# Autodesk Inventor assembly: euph cart bottom
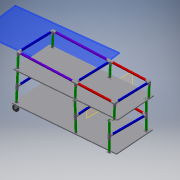
[picture p0: Inventor's stored thumbnail of the model, 180x180]
Saved by Autodesk Inventor 2018.2 (Build 222227000, 227)
## iProperties
Created: 2018-02-07
Part Number: euph cart bottom
Document SubType Name: Assembly
Designer: owner
Author: owner
## Documents named in this file (12)
- Z:\The Pickle\Final Carts\Euph Cart\euph cart bottom.iam
- Z:\The Pickle\Final Carts\Euph Cart\Plywood Base.ipt
- Z:\The Pickle\Inventor Pipe Parts\Formufit Fittings\4-way Tee 1 Inch.ipt
- Z:\The Pickle\Inventor Pipe Parts\Formufit Fittings\Tee 1 Inch.ipt
- Z:\The Pickle\Inventor Pipe Parts\Formufit Fittings\Wood Mount 1 Inch.ipt
- Z:\The Pickle\Final Carts\Euph Cart\Pipe 1.ipt
- Z:\The Pickle\Final Carts\Euph Cart\Pipe 2.ipt
- Z:\The Pickle\Final Carts\Euph Cart\Pipe 3.ipt
- Z:\The Pickle\Final Carts\WHEELS.ipt
- Z:\The Pickle\Final Carts\Mellie Cart\Pipe 4.ipt
- Z:\The Pickle\Inventor Pipe Parts\Formufit Fittings\5-way 1 Inch.ipt
- Z:\The Pickle\Inventor Pipe Parts\Formufit Fittings\3-way 90 1 Inch.ipt
## Components (65 placed, 11 different names)
1. Tee 1 Inch:4 — Insert:41, Insert:42, Insert:45
2. Pipe 1:2 — Insert:51, Insert:65
3. Plywood Base:2 — Mate:3, Flush:4, Flush:5, Flush:6, Tangent:6, Tangent:7, Flush:18, Flush:19, Mate:7
4. 4-way Tee 1 Inch:5
5. Wood Mount 1 Inch:9 — Tangent:6, Tangent:7, Flush:12, Mate:7
6. Wood Mount 1 Inch:10 — Flush:13
7. Wood Mount 1 Inch:11 — Flush:14
8. Wood Mount 1 Inch:12 — Flush:15
9. Pipe 1:3 — Insert:42
10. Pipe 2:4 — Insert:50
11. Pipe 3:9 — Insert:49
12. Pipe 3:10
13. Pipe 3:11 — Insert:41
14. Pipe 3:12 — Insert:72
15. Pipe 3:13 — Insert:52, Insert:73
16. Pipe 3:14 — Insert:66, Insert:74
17. Pipe 3:15 — Insert:45, Insert:71, Mate:6
18. Pipe 3:16 — Insert:70
19. WHEELS:1 — Flush:2, Flush:3, Mate:3, Flush:4, Flush:5, Flush:7
20. WHEELS:2 — Flush:2, Flush:6, Flush:7, Flush:11
21. WHEELS:4 — Flush:3, Flush:11
22. Pipe 4:3 — Insert:118, Insert:119
23. Pipe 4:7 — Insert:58
24. Pipe 1:11 — Insert:57, Insert:67
25. Wood Mount 1 Inch:13 — Insert:63, Flush:17
26. Wood Mount 1 Inch:14 — Insert:64, Flush:16
27. Wood Mount 1 Inch:15 — Insert:72, Flush:13
28. Wood Mount 1 Inch:16 — Insert:73, Flush:15
29. Wood Mount 1 Inch:17 — Insert:71, Flush:12, Mate:4
30. Wood Mount 1 Inch:18 — Insert:74, Flush:14
31. 5-way 1 Inch:1 — Insert:49, Insert:50, Insert:51, Insert:52
32. 4-way Tee 1 Inch:6 — Insert:57, Insert:58, Insert:61, Insert:62
33. Pipe 3:17 — Insert:63, Insert:68
34. Pipe 3:18 — Insert:69, Insert:75
35. Pipe 3:23 — Insert:61, Insert:64
36. Pipe 3:26 — Insert:62, Insert:76
37. Tee 1 Inch:5 — Insert:65, Insert:66, Insert:70
38. Tee 1 Inch:6 — Insert:67, Insert:68, Insert:69
39. Plywood Base:3 — Mate:4, Flush:18, Flush:19, Mate:5
40. Wood Mount 1 Inch:19 — Insert:75, Flush:17
41. Wood Mount 1 Inch:20 — Insert:76, Flush:16
42. Pipe 2:5 — Insert:105, Insert:109
43. Pipe 1:12 — Insert:108, Insert:111
44. Wood Mount 1 Inch:21 — Mate:5
45. Wood Mount 1 Inch:22
46. Wood Mount 1 Inch:23
47. Wood Mount 1 Inch:24
48. Pipe 1:13 — Insert:101, Insert:103
49. Pipe 2:6 — Insert:104, Insert:106
50. Pipe 3:27 — Insert:107
51. Pipe 3:28 — Insert:102
52. Pipe 3:29 — Mate:6, Insert:100
53. Pipe 3:34 — Insert:110
54. Pipe 4:8 — Insert:112, Insert:113
55. Pipe 1:14 — Insert:115, Insert:117
56. Wood Mount 1 Inch:25
57. Wood Mount 1 Inch:26
58. Pipe 3:35 — Insert:116
59. Pipe 3:37 — Insert:114
60. 4-way Tee 1 Inch:9 — Insert:106, Insert:107, Insert:108, Insert:112
61. 4-way Tee 1 Inch:10 — Insert:109, Insert:110, Insert:111, Insert:118
62. 3-way 90 1 Inch:1 — Insert:102, Insert:103, Insert:104
63. 3-way 90 1 Inch:2 — Insert:113, Insert:114, Insert:115
64. 3-way 90 1 Inch:3 — Insert:116, Insert:117, Insert:119
65. 3-way 90 1 Inch:4 — Insert:100, Insert:101, Insert:105
## Relationships (81: Insert 59, Flush 15, Mate 5, Tangent 2)
- [Insert]: Wood Mount 1 Inch:11 ↔ Pipe 3:16
- [Insert]: 4-way Tee 1 Inch:5 ↔ Pipe 1:3
- [Insert]: 4-way Tee 1 Inch:5 ↔ Pipe 2:4
- [Insert]: 4-way Tee 1 Inch:5 ↔ Pipe 3:10
- [Insert]: Wood Mount 1 Inch:12 ↔ Pipe 3:9
- [Insert]: Wood Mount 1 Inch:10 ↔ Pipe 3:10
- [Insert]: Wood Mount 1 Inch:9 ↔ Pipe 3:11
- [Insert]: 4-way Tee 1 Inch:5 ↔ Pipe 3:12
- Insert:41: Tee 1 Inch:4 ↔ Pipe 3:11
- Insert:42: Tee 1 Inch:4 ↔ Pipe 1:3
- Insert:45: Tee 1 Inch:4 ↔ Pipe 3:15
- Flush:2: WHEELS:1 ↔ WHEELS:2
- Flush:3: WHEELS:1 ↔ WHEELS:4
- Mate:3: Plywood Base:2 ↔ WHEELS:1
- Flush:4 (12.7 mm): Plywood Base:2 ↔ WHEELS:1
- Flush:5 (12.7 mm): Plywood Base:2 ↔ WHEELS:1
- Flush:6 (12.7 mm): Plywood Base:2 ↔ WHEELS:2
- Flush:7: WHEELS:1 ↔ WHEELS:2
- Flush:11: WHEELS:2 ↔ WHEELS:4
- Tangent:6: Plywood Base:2 ↔ Wood Mount 1 Inch:9
- Tangent:7: Plywood Base:2 ↔ Wood Mount 1 Inch:9
- Insert:49: Pipe 3:9 ↔ 5-way 1 Inch:1
- Insert:50: Pipe 2:4 ↔ 5-way 1 Inch:1
- Insert:51: Pipe 1:2 ↔ 5-way 1 Inch:1
- Insert:52: Pipe 3:13 ↔ 5-way 1 Inch:1
- Insert:57: Pipe 1:11 ↔ 4-way Tee 1 Inch:6
- Insert:58: Pipe 4:7 ↔ 4-way Tee 1 Inch:6
- Insert:61: 4-way Tee 1 Inch:6 ↔ Pipe 3:23
- Insert:62: 4-way Tee 1 Inch:6 ↔ Pipe 3:26
- Insert:63: Wood Mount 1 Inch:13 ↔ Pipe 3:17
- Insert:64: Wood Mount 1 Inch:14 ↔ Pipe 3:23
- Insert:65: Pipe 1:2 ↔ Tee 1 Inch:5
- Insert:66: Pipe 3:14 ↔ Tee 1 Inch:5
- Insert:67: Pipe 1:11 ↔ Tee 1 Inch:6
- Insert:68: Pipe 3:17 ↔ Tee 1 Inch:6
- Insert:69: Pipe 3:18 ↔ Tee 1 Inch:6
- Insert:70: Pipe 3:16 ↔ Tee 1 Inch:5
- Insert:71: Pipe 3:15 ↔ Wood Mount 1 Inch:17
- Insert:72: Pipe 3:12 ↔ Wood Mount 1 Inch:15
- Insert:73: Pipe 3:13 ↔ Wood Mount 1 Inch:16
- Insert:74: Pipe 3:14 ↔ Wood Mount 1 Inch:18
- Insert:75: Pipe 3:18 ↔ Wood Mount 1 Inch:19
- Insert:76: Pipe 3:26 ↔ Wood Mount 1 Inch:20
- Flush:12: Wood Mount 1 Inch:9 ↔ Wood Mount 1 Inch:17
- Flush:13: Wood Mount 1 Inch:10 ↔ Wood Mount 1 Inch:15
- Flush:14: Wood Mount 1 Inch:11 ↔ Wood Mount 1 Inch:18
- Flush:15: Wood Mount 1 Inch:12 ↔ Wood Mount 1 Inch:16
- Flush:16: Wood Mount 1 Inch:14 ↔ Wood Mount 1 Inch:20
- Flush:17: Wood Mount 1 Inch:13 ↔ Wood Mount 1 Inch:19
- Mate:4: Wood Mount 1 Inch:17 ↔ Plywood Base:3
- Flush:18: Plywood Base:2 ↔ Plywood Base:3
- Flush:19: Plywood Base:2 ↔ Plywood Base:3
- [Insert]: Wood Mount 1 Inch:23 ↔ Pipe 3:34
- [Insert]: Wood Mount 1 Inch:24 ↔ Pipe 3:27
- [Insert]: Wood Mount 1 Inch:22 ↔ Pipe 3:28
- [Insert]: Wood Mount 1 Inch:21 ↔ Pipe 3:29
- [Insert]: Wood Mount 1 Inch:25 ↔ Pipe 3:35
- [Insert]: Wood Mount 1 Inch:26 ↔ Pipe 3:37
- Mate:5: Plywood Base:3 ↔ Wood Mount 1 Inch:21
- Mate:6: Pipe 3:15 ↔ Pipe 3:29
- Insert:100: Pipe 3:29 ↔ 3-way 90 1 Inch:4
- Insert:101: Pipe 1:13 ↔ 3-way 90 1 Inch:4
- Insert:102: Pipe 3:28 ↔ 3-way 90 1 Inch:1
- Insert:103: Pipe 1:13 ↔ 3-way 90 1 Inch:1
- Insert:104: Pipe 2:6 ↔ 3-way 90 1 Inch:1
- Insert:105: Pipe 2:5 ↔ 3-way 90 1 Inch:4
- Insert:106: Pipe 2:6 ↔ 4-way Tee 1 Inch:9
- Insert:107: Pipe 3:27 ↔ 4-way Tee 1 Inch:9
- Insert:108: Pipe 1:12 ↔ 4-way Tee 1 Inch:9
- Insert:109: Pipe 2:5 ↔ 4-way Tee 1 Inch:10
- Insert:110: Pipe 3:34 ↔ 4-way Tee 1 Inch:10
- Insert:111: Pipe 1:12 ↔ 4-way Tee 1 Inch:10
- Insert:112: Pipe 4:8 ↔ 4-way Tee 1 Inch:9
- Insert:113: Pipe 4:8 ↔ 3-way 90 1 Inch:2
- Insert:114: Pipe 3:37 ↔ 3-way 90 1 Inch:2
- Insert:115: Pipe 1:14 ↔ 3-way 90 1 Inch:2
- Insert:116: Pipe 3:35 ↔ 3-way 90 1 Inch:3
- Insert:117: Pipe 1:14 ↔ 3-way 90 1 Inch:3
- Insert:118: Pipe 4:3 ↔ 4-way Tee 1 Inch:10
- Insert:119: Pipe 4:3 ↔ 3-way 90 1 Inch:3
- Mate:7: Plywood Base:2 ↔ Wood Mount 1 Inch:9
## Named parameters: d21_d12 = 0 mm, d23_d14 = 0 mm, d24_d15 = 0 mm, d25_d16 = 0 mm, d28_d19 = 0 mm, d32_d3 = 0 mm, d37_d8 = 0 mm, d38_d9 = 0 mm, d182_d156 = 0 mm, d205_d155 = 0 mm, d216_d23_d14 = 0 mm, d217_d24_d15 = 0 mm, d218_d25_d16 = 0 mm, d220_d32_d3 = 0 mm
